# Autodesk Inventor assembly: G60
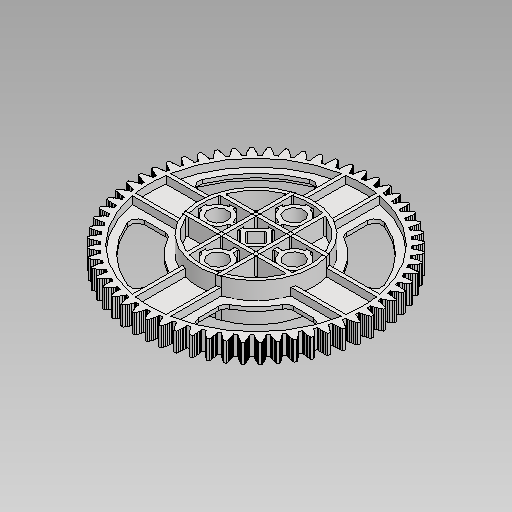
[picture p0: Inventor's stored thumbnail of the model, 512x512]
Saved by Autodesk Inventor 2020 (Build 240168000, 168)
## iProperties
Created: 2019-05-06
Part Number: G60
Document SubType Name: Assembly
Designer: Varga Daniel
Author: Varga Daniel
## Documents named in this file (3)
- C:\!_Dani\!_cloud\OneDrive\!_munka\Revolution\StructuralParts\Gears\G60.iam
- C:\!_Dani\!_cloud\OneDrive\!_munka\Revolution\StructuralParts\Gears\Gear central part.iam
- C:\!_Dani\!_cloud\OneDrive\!_munka\Revolution\StructuralParts\Gears\gear60_tooth.ipt
## Components (2 placed, 2 different names)
1. Gear central part:1 [sub-assembly] — Mate:1, Mate:2, Flush:1, Mate:3, Mate:4, Flush:2
2. gear60_tooth:1 — Mate:1, Mate:2, Flush:1
## Relationships (6: Mate 4, Flush 2)
- Mate:1: Gear central part:1 ↔ gear60_tooth:1
- Mate:2: Gear central part:1 ↔ gear60_tooth:1
- Flush:1: Gear central part:1 ↔ gear60_tooth:1
- Mate:3: Gear central part:1
- Mate:4: Gear central part:1
- Flush:2: Gear central part:1
